# Autodesk Inventor assembly: ROBOT_5GDL
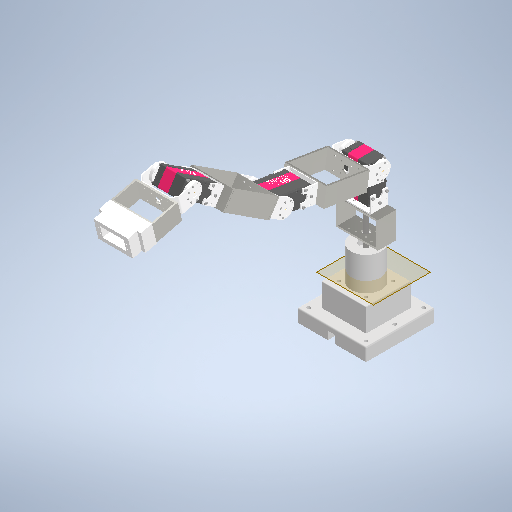
[picture p0: Inventor's stored thumbnail of the model, 512x512]
Saved by Autodesk Inventor 2025.1 (Build 291241000, 241)
## iProperties
Created: 2024-12-02
Part Number: ROBOT_5GDL
Document SubType Name: Assembly
Designer: Cristhian Vigo
Author: Cristhian Vigo
## Documents named in this file (20)
- D:\CRISTHIAN\universidad\ciclo 8\Robótica\PROYECTO\Modelo\ROBOT_5GDL\ROBOT_5GDL.iam
- D:\CRISTHIAN\universidad\ciclo 8\Robótica\PROYECTO\Modelo\ROBOT_5GDL\base.ipt
- D:\CRISTHIAN\universidad\ciclo 8\Robótica\PROYECTO\Modelo\ROBOT_5GDL\Servo.ipt
- D:\CRISTHIAN\universidad\ciclo 8\Robótica\PROYECTO\Modelo\ROBOT_5GDL\base giratoria.ipt
- D:\CRISTHIAN\universidad\ciclo 8\Robótica\PROYECTO\Modelo\ROBOT_5GDL\DIN_EN_ISO_4762_M2,5x5.ipt v2.ipt
- D:\CRISTHIAN\universidad\ciclo 8\Robótica\PROYECTO\Modelo\ROBOT_5GDL\DIN_EN_ISO_4762_M2,5x25.ipt v2.ipt
- D:\CRISTHIAN\universidad\ciclo 8\Robótica\PROYECTO\Modelo\ROBOT_5GDL\engranaje recto servo.ipt
- D:\CRISTHIAN\universidad\ciclo 8\Robótica\PROYECTO\Modelo\ROBOT_5GDL\rodamiento.ipt
- D:\CRISTHIAN\universidad\ciclo 8\Robótica\PROYECTO\Modelo\ROBOT_5GDL\Soporte 1.ipt
- D:\CRISTHIAN\universidad\ciclo 8\Robótica\PROYECTO\Modelo\ROBOT_5GDL\Soporte 2.ipt
- D:\CRISTHIAN\universidad\ciclo 8\Robótica\PROYECTO\Modelo\ROBOT_5GDL\Screw 3 v1.ipt
- D:\CRISTHIAN\universidad\ciclo 8\Robótica\PROYECTO\Modelo\ROBOT_5GDL\Eslabón3.iam
- D:\CRISTHIAN\universidad\ciclo 8\Robótica\PROYECTO\Modelo\ROBOT_5GDL\Eslabón4.iam
- D:\CRISTHIAN\universidad\ciclo 8\Robótica\PROYECTO\Modelo\ROBOT_5GDL\NEMA 23 - 41mm\Inventor\NEMA 23 - 41mm.iam
- D:\CRISTHIAN\universidad\ciclo 8\Robótica\PROYECTO\Modelo\ROBOT_5GDL\Eslabón2.iam
- D:\CRISTHIAN\universidad\ciclo 8\Robótica\PROYECTO\Modelo\ROBOT_5GDL\Eslabon1.ipt
- D:\CRISTHIAN\universidad\ciclo 8\Robótica\PROYECTO\Modelo\ROBOT_5GDL\Eje8mm.ipt
- D:\CRISTHIAN\universidad\ciclo 8\Robótica\PROYECTO\Modelo\ROBOT_5GDL\Base_servo_efector.ipt
- DIN_EN_ISO_4762_M2,5x5.ipt
- DIN_EN_ISO_4762_M2,5x25.ipt
## Components (89 placed, 17 different names)
1. base:1
2. Servo:1
3. base giratoria:1
4. DIN_EN_ISO_4762_M2,5x5.ipt v2:1
5. DIN_EN_ISO_4762_M2,5x25.ipt v2:1
6. engranaje recto servo:1
7. rodamiento:1
8. Soporte 1:1 — Flush:1, Flush:2, Mate:7
9. Soporte 2:1 — Flush:7, Flush:8, Mate:16
10. DIN_EN_ISO_4762_M2,5x5.ipt v2:2
11. DIN_EN_ISO_4762_M2,5x5.ipt v2:3
12. DIN_EN_ISO_4762_M2,5x5.ipt v2:4
13. DIN_EN_ISO_4762_M2,5x5.ipt v2:5
14. DIN_EN_ISO_4762_M2,5x5.ipt v2:6
15. DIN_EN_ISO_4762_M2,5x25.ipt v2:2
16. DIN_EN_ISO_4762_M2,5x25.ipt v2:3
17. DIN_EN_ISO_4762_M2,5x25.ipt v2:4
18. Screw 3 v1:1
19. Screw 3 v1:2
20. Screw 3 v1:3
21. Screw 3 v1:4
22. Screw 3 v1:5
23. Screw 3 v1:6
24. Screw 3 v1:7
25. Screw 3 v1:8
26. Screw 3 v1:9
27. Screw 3 v1:10
28. Eslabón3:1 [sub-assembly] — Flush:1, Flush:2, Mate:7, Mate:14, Flush:3, Flush:4
29. base:2
30. Servo:2
31. base giratoria:2
32. DIN_EN_ISO_4762_M2,5x5.ipt v2:7
33. DIN_EN_ISO_4762_M2,5x25.ipt v2:5
34. engranaje recto servo:2
35. rodamiento:2
36. Soporte 1:2 — Flush:5, Flush:6, Mate:15
37. Soporte 2:2 — Mate:14, Flush:3, Flush:4
38. DIN_EN_ISO_4762_M2,5x5.ipt v2:8
39. DIN_EN_ISO_4762_M2,5x5.ipt v2:9
40. DIN_EN_ISO_4762_M2,5x5.ipt v2:10
41. DIN_EN_ISO_4762_M2,5x5.ipt v2:11
42. DIN_EN_ISO_4762_M2,5x5.ipt v2:12
43. DIN_EN_ISO_4762_M2,5x25.ipt v2:6
44. DIN_EN_ISO_4762_M2,5x25.ipt v2:7
45. DIN_EN_ISO_4762_M2,5x25.ipt v2:8
46. Screw 3 v1:11
47. Screw 3 v1:12
48. Screw 3 v1:13
49. Screw 3 v1:14
50. Screw 3 v1:15
51. Screw 3 v1:16
52. Screw 3 v1:17
53. Screw 3 v1:18
54. Screw 3 v1:19
55. Screw 3 v1:20
56. Eslabón4:1 [sub-assembly] — Flush:5, Flush:6, Mate:15, Mate:26, Flush:15, Flush:16
57. NEMA 23 - 41mm:1 [sub-assembly] — Insert:106, Insert:107
58. Eslabón2:1 [sub-assembly] — Flush:7, Flush:8, Mate:16, Flush:9, Flush:10, Mate:23
59. base:3
60. Servo:3
61. base giratoria:3
62. DIN_EN_ISO_4762_M2,5x5.ipt v2:13
63. DIN_EN_ISO_4762_M2,5x25.ipt v2:9
64. engranaje recto servo:3
65. rodamiento:3
66. Soporte 1:3 — Flush:9, Flush:10, Mate:23
67. Soporte 2:3 — Mate:27, Flush:17, Flush:18
68. DIN_EN_ISO_4762_M2,5x5.ipt v2:14
69. DIN_EN_ISO_4762_M2,5x5.ipt v2:15
70. DIN_EN_ISO_4762_M2,5x5.ipt v2:16
71. DIN_EN_ISO_4762_M2,5x5.ipt v2:17
72. DIN_EN_ISO_4762_M2,5x5.ipt v2:18
73. DIN_EN_ISO_4762_M2,5x25.ipt v2:10
74. DIN_EN_ISO_4762_M2,5x25.ipt v2:11
75. DIN_EN_ISO_4762_M2,5x25.ipt v2:12
76. Screw 3 v1:21
77. Screw 3 v1:22
78. Screw 3 v1:23
79. Screw 3 v1:24
80. Screw 3 v1:25
81. Screw 3 v1:26
82. Screw 3 v1:27
83. Screw 3 v1:28
84. Screw 3 v1:29
85. Screw 3 v1:30
86. Eslabon1:1 — Insert:106, Insert:107, Insert:109
87. Eje8mm:1 — Insert:109, Insert:110
88. Base_servo_efector:1 — Mate:26, Flush:15, Flush:16
89. Eslabón4:2 [sub-assembly] — Mate:27, Flush:17, Flush:18, Insert:110
## Relationships (115: Insert 76, Mate 25, Flush 14)
- [Mate]: Servo:1 ↔ Soporte 2:1
- [Mate]: Servo:1 ↔ Soporte 2:1
- [Mate]: Servo:1 ↔ Soporte 2:1
- [Insert]: DIN_EN_ISO_4762_M2,5x5.ipt v2:1 ↔ Soporte 2:1
- [Insert]: Soporte 2:1 ↔ DIN_EN_ISO_4762_M2,5x5.ipt v2:2
- [Insert]: Soporte 2:1 ↔ DIN_EN_ISO_4762_M2,5x5.ipt v2:3
- [Insert]: Soporte 2:1 ↔ DIN_EN_ISO_4762_M2,5x5.ipt v2:5
- [Insert]: Soporte 2:1 ↔ DIN_EN_ISO_4762_M2,5x5.ipt v2:4
- [Insert]: Soporte 2:1 ↔ DIN_EN_ISO_4762_M2,5x5.ipt v2:6
- [Insert]: base:1 ↔ rodamiento:1
- [Insert]: base:1 ↔ Servo:1
- [Insert]: Servo:1 ↔ engranaje recto servo:1
- [Insert]: base giratoria:1 ↔ engranaje recto servo:1
- [Insert]: Servo:1 ↔ DIN_EN_ISO_4762_M2,5x25.ipt v2:1
- [Insert]: Servo:1 ↔ DIN_EN_ISO_4762_M2,5x25.ipt v2:4
- [Insert]: Servo:1 ↔ DIN_EN_ISO_4762_M2,5x25.ipt v2:2
- [Insert]: Servo:1 ↔ DIN_EN_ISO_4762_M2,5x25.ipt v2:3
- [Mate]: base giratoria:1 ↔ Soporte 1:1
- [Mate]: base giratoria:1 ↔ Soporte 1:1
- [Mate]: base:1 ↔ Soporte 1:1
- [Insert]: Soporte 1:1 ↔ Screw 3 v1:4
- [Insert]: Soporte 1:1 ↔ Screw 3 v1:5
- [Insert]: Soporte 1:1 ↔ Screw 3 v1:3
- [Insert]: Soporte 1:1 ↔ Screw 3 v1:2
- [Insert]: Soporte 1:1 ↔ Screw 3 v1:1
- [Insert]: Soporte 1:1 ↔ Screw 3 v1:7
- [Insert]: Soporte 1:1 ↔ Screw 3 v1:6
- [Insert]: Soporte 1:1 ↔ Screw 3 v1:8
- [Insert]: Soporte 1:1 ↔ Screw 3 v1:10
- [Insert]: Soporte 1:1 ↔ Screw 3 v1:9
- Flush:1: Soporte 1:1 ↔ Eslabón3:1
- Flush:2 (-1 mm): Soporte 1:1 ↔ Eslabón3:1
- Mate:7: Soporte 1:1 ↔ Eslabón3:1
- [Mate]: Servo:2 ↔ Soporte 2:2
- [Mate]: Servo:2 ↔ Soporte 2:2
- [Mate]: Servo:2 ↔ Soporte 2:2
- [Insert]: DIN_EN_ISO_4762_M2,5x5.ipt v2:7 ↔ Soporte 2:2
- [Insert]: Soporte 2:2 ↔ DIN_EN_ISO_4762_M2,5x5.ipt v2:8
- [Insert]: Soporte 2:2 ↔ DIN_EN_ISO_4762_M2,5x5.ipt v2:9
- [Insert]: Soporte 2:2 ↔ DIN_EN_ISO_4762_M2,5x5.ipt v2:11
- [Insert]: Soporte 2:2 ↔ DIN_EN_ISO_4762_M2,5x5.ipt v2:10
- [Insert]: Soporte 2:2 ↔ DIN_EN_ISO_4762_M2,5x5.ipt v2:12
- [Insert]: base:2 ↔ rodamiento:2
- [Insert]: base:2 ↔ Servo:2
- [Insert]: Servo:2 ↔ engranaje recto servo:2
- [Insert]: base giratoria:2 ↔ engranaje recto servo:2
- [Insert]: Servo:2 ↔ DIN_EN_ISO_4762_M2,5x25.ipt v2:5
- [Insert]: Servo:2 ↔ DIN_EN_ISO_4762_M2,5x25.ipt v2:8
- [Insert]: Servo:2 ↔ DIN_EN_ISO_4762_M2,5x25.ipt v2:6
- [Insert]: Servo:2 ↔ DIN_EN_ISO_4762_M2,5x25.ipt v2:7
- [Mate]: base giratoria:2 ↔ Soporte 1:2
- [Mate]: base giratoria:2 ↔ Soporte 1:2
- [Mate]: base:2 ↔ Soporte 1:2
- [Insert]: Soporte 1:2 ↔ Screw 3 v1:14
- [Insert]: Soporte 1:2 ↔ Screw 3 v1:15
- [Insert]: Soporte 1:2 ↔ Screw 3 v1:13
- [Insert]: Soporte 1:2 ↔ Screw 3 v1:12
- [Insert]: Soporte 1:2 ↔ Screw 3 v1:11
- [Insert]: Soporte 1:2 ↔ Screw 3 v1:17
- [Insert]: Soporte 1:2 ↔ Screw 3 v1:16
- [Insert]: Soporte 1:2 ↔ Screw 3 v1:18
- [Insert]: Soporte 1:2 ↔ Screw 3 v1:20
- [Insert]: Soporte 1:2 ↔ Screw 3 v1:19
- Mate:14: Eslabón3:1 ↔ Soporte 2:2
- Flush:3 (1 mm): Eslabón3:1 ↔ Soporte 2:2
- Flush:4 (8 mm): Eslabón3:1 ↔ Soporte 2:2
- Flush:5: Soporte 1:2 ↔ Eslabón4:1
- Flush:6 (-1 mm): Soporte 1:2 ↔ Eslabón4:1
- Mate:15: Soporte 1:2 ↔ Eslabón4:1
- Flush:7 (8 mm): Soporte 2:1 ↔ Eslabón2:1
- Flush:8 (-1 mm): Soporte 2:1 ↔ Eslabón2:1
- Mate:16: Soporte 2:1 ↔ Eslabón2:1
- [Mate]: Servo:3 ↔ Soporte 2:3
- [Mate]: Servo:3 ↔ Soporte 2:3
- [Mate]: Servo:3 ↔ Soporte 2:3
- [Insert]: DIN_EN_ISO_4762_M2,5x5.ipt v2:13 ↔ Soporte 2:3
- [Insert]: Soporte 2:3 ↔ DIN_EN_ISO_4762_M2,5x5.ipt v2:14
- [Insert]: Soporte 2:3 ↔ DIN_EN_ISO_4762_M2,5x5.ipt v2:15
- [Insert]: Soporte 2:3 ↔ DIN_EN_ISO_4762_M2,5x5.ipt v2:17
- [Insert]: Soporte 2:3 ↔ DIN_EN_ISO_4762_M2,5x5.ipt v2:16
- [Insert]: Soporte 2:3 ↔ DIN_EN_ISO_4762_M2,5x5.ipt v2:18
- [Insert]: base:3 ↔ rodamiento:3
- [Insert]: base:3 ↔ Servo:3
- [Insert]: Servo:3 ↔ engranaje recto servo:3
- [Insert]: base giratoria:3 ↔ engranaje recto servo:3
- [Insert]: Servo:3 ↔ DIN_EN_ISO_4762_M2,5x25.ipt v2:9
- [Insert]: Servo:3 ↔ DIN_EN_ISO_4762_M2,5x25.ipt v2:12
- [Insert]: Servo:3 ↔ DIN_EN_ISO_4762_M2,5x25.ipt v2:10
- [Insert]: Servo:3 ↔ DIN_EN_ISO_4762_M2,5x25.ipt v2:11
- [Mate]: base giratoria:3 ↔ Soporte 1:3
- [Mate]: base giratoria:3 ↔ Soporte 1:3
- [Mate]: base:3 ↔ Soporte 1:3
- [Insert]: Soporte 1:3 ↔ Screw 3 v1:24
- [Insert]: Soporte 1:3 ↔ Screw 3 v1:25
- [Insert]: Soporte 1:3 ↔ Screw 3 v1:23
- [Insert]: Soporte 1:3 ↔ Screw 3 v1:22
- [Insert]: Soporte 1:3 ↔ Screw 3 v1:21
- [Insert]: Soporte 1:3 ↔ Screw 3 v1:27
- [Insert]: Soporte 1:3 ↔ Screw 3 v1:26
- [Insert]: Soporte 1:3 ↔ Screw 3 v1:28
- [Insert]: Soporte 1:3 ↔ Screw 3 v1:30
- [Insert]: Soporte 1:3 ↔ Screw 3 v1:29
- Flush:9: Eslabón2:1 ↔ Soporte 1:3
- Flush:10 (-1 mm): Eslabón2:1 ↔ Soporte 1:3
- Mate:23: Eslabón2:1 ↔ Soporte 1:3
- Insert:106: NEMA 23 - 41mm:1 ↔ Eslabon1:1
- Insert:107: NEMA 23 - 41mm:1 ↔ Eslabon1:1
- Insert:109 (-28 mm): Eslabon1:1 ↔ Eje8mm:1
- Mate:26: Eslabón4:1 ↔ Base_servo_efector:1
- Flush:15: Eslabón4:1 ↔ Base_servo_efector:1
- Flush:16 (-1.5 mm): Eslabón4:1 ↔ Base_servo_efector:1
- Mate:27: Soporte 2:3 ↔ Eslabón4:2
- Flush:17 (-7.5 mm): Soporte 2:3 ↔ Eslabón4:2
- Flush:18 (-1 mm): Soporte 2:3 ↔ Eslabón4:2
- Insert:110: Eje8mm:1 ↔ Eslabón4:2
## Named parameters: d0_d4 = 0 mm, d1_d5 = 0 mm, d2_d6 = 0 mm, d16_d25 = 0 mm, d17_d26 = 0 mm, d18_d27 = 0 mm, d19_d28 = 0 mm, d20_d29 = 0 mm, d56_d0_d4 = 0 mm, d57_d1_d5 = 0 mm, d58_d2_d6 = 0 mm, d59_d42 = 0 mm, d60_d43 = 0 mm, d61_d44 = 0 mm, d62_d45 = 0 mm, d63_d46 = 0 mm, d64_d7 = 0 mm, d65_d8 = 0 mm, d66_d9 = 0 mm, d67_d10 = 0 mm, d68_d11 = 0 mm, d69_d12 = 0 mm, d70_d14 = 0 mm, d71_d15 = 0 mm, d72_d16_d25 = 0 mm, d73_d17_d26 = 0 mm, d74_d18_d27 = 0 mm, d75_d19_d28 = 0 mm, d76_d20_d29 = 0 mm, d77_d30 = 0 mm, d78_d31 = 0 mm, d79_d32 = 0 mm, d80_d33 = 0 mm, d81_d34 = 0 mm, d82_d35 = 0 mm, d83_d37 = 0 mm, d84_d39 = 0 mm, d85_d41 = 0 mm, d95_d0_d4 = 0 mm, d96_d1_d5 = 0 mm, d97_d2_d6 = 0 mm, d98_d42 = 0 mm, d99_d43 = 0 mm, d100_d44 = 0 mm, d101_d45 = 0 mm, d102_d46 = 0 mm, d103_d7 = 0 mm, d104_d8 = 0 mm, d105_d9 = 0 mm, d106_d10 = 0 mm, d107_d11 = 0 mm, d108_d12 = 0 mm, d109_d14 = 0 mm, d110_d15 = 0 mm, d111_d16_d25 = 0 mm, d112_d17_d26 = 0 mm, d113_d18_d27 = 0 mm, d114_d19_d28 = 0 mm, d115_d20_d29 = 0 mm, d116_d30 = 0 mm, d117_d31 = 0 mm, d118_d32 = 0 mm, d119_d33 = 0 mm, d120_d34 = 0 mm, d121_d35 = 0 mm, d122_d37 = 0 mm, d123_d39 = 0 mm, d124_d41 = 0 mm
